# Autodesk Inventor assembly: cover_back_left
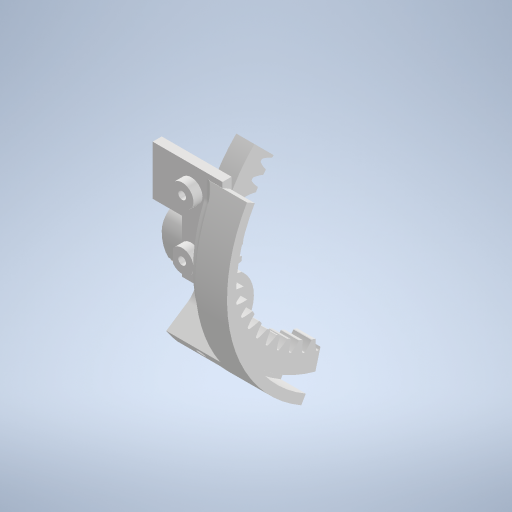
[picture p0: Inventor's stored thumbnail of the model, 512x512]
Saved by Autodesk Inventor 2024.1 (Build 281209000, 209)
## iProperties
Created: 2025-01-10
Part Number: cover_back_left
Document SubType Name: Assembly
Designer: hibik
Author: hibik
## Documents named in this file (3)
- C:\Users\hibik\Documents\Robomech\RESCUE\ORCA\hard\camera\cover_back_left.iam
- C:\Users\hibik\Documents\Robomech\RESCUE\ORCA\hard\camera\cover_back_left_base.ipt
- C:\Users\hibik\Documents\Robomech\RESCUE\ORCA\hard\camera\cover_back_left_gear.ipt
## Components (2 placed, 2 different names)
1. cover_back_left_base:1 — 挿入:1
2. cover_back_left_gear:1 — 挿入:1, 角度:1
## Relationships (2: Insert 1, Angle 1)
- 挿入:1 [Insert]: cover_back_left_base:1 ↔ cover_back_left_gear:1
- 角度:1 [Angle] (45 deg): cover_back_left_gear:1
